# Autodesk Inventor assembly: 53
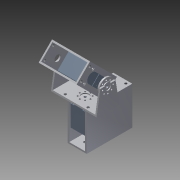
[picture p0: Inventor's stored thumbnail of the model, 180x180]
Saved by Autodesk Inventor 2013 (Build 170138000, 138)
## iProperties
Created: 2014-04-04
Part Number: 53
Document SubType Name: Assembly
Designer: andou
Author: andou
Title: Head
## Documents named in this file (7)
- C:\Users\andou\Documents\GitHub\Robotics-Project\design\RoboticsProject\project_4\Head.iam
- C:\Users\andou\Documents\GitHub\Robotics-Project\design\RoboticsProject\project_4\Long_Serial_Case.ipt
- C:\Users\andou\Documents\GitHub\Robotics-Project\design\RoboticsProject\project_4\Generic Parts\KRS-2542HV.ipt
- C:\Users\andou\Documents\GitHub\Robotics-Project\design\RoboticsProject\project_4\Generic Parts\Low_Height_Horn.ipt
- C:\Users\andou\Documents\GitHub\Robotics-Project\design\RoboticsProject\project_4\Complete_data\Bracket.ipt
- C:\Users\andou\Documents\GitHub\Robotics-Project\design\RoboticsProject\project_4\Complete_data\Serial_Case.ipt
- C:\Users\andou\Documents\GitHub\Robotics-Project\design\RoboticsProject\project_4\Complete_data\Free_Horn.iam
## Components (8 placed, 6 different names)
1. Long_Serial_Case:1 — 挿入:1, 挿入:2
2. KRS-2542HV:1 — 挿入:1, 挿入:2, 挿入:3
3. Low_Height_Horn:1 — 挿入:3, 挿入:7, 挿入:8
4. Bracket:1 — 挿入:7, 挿入:8, 挿入:10, 挿入:11, 挿入:12
5. Serial_Case:1 — 挿入:5, 挿入:6, 挿入:9
6. KRS-2542HV:2 — 挿入:4, 挿入:5, 挿入:6
7. Low_Height_Horn:2 — 挿入:4, 挿入:10, 挿入:11
8. Free_Horn:1 [sub-assembly] — 挿入:9, 挿入:12
## Relationships (12: Insert 12)
- 挿入:1 [Insert]: Long_Serial_Case:1 ↔ KRS-2542HV:1
- 挿入:2 [Insert]: Long_Serial_Case:1 ↔ KRS-2542HV:1
- 挿入:3 [Insert]: KRS-2542HV:1 ↔ Low_Height_Horn:1
- 挿入:4 [Insert]: KRS-2542HV:2 ↔ Low_Height_Horn:2
- 挿入:5 [Insert]: Serial_Case:1 ↔ KRS-2542HV:2
- 挿入:6 [Insert]: Serial_Case:1 ↔ KRS-2542HV:2
- 挿入:7 [Insert]: Low_Height_Horn:1 ↔ Bracket:1
- 挿入:8 [Insert]: Low_Height_Horn:1 ↔ Bracket:1
- 挿入:9 [Insert]: Serial_Case:1 ↔ Free_Horn:1
- 挿入:10 [Insert]: Bracket:1 ↔ Low_Height_Horn:2
- 挿入:11 [Insert]: Bracket:1 ↔ Low_Height_Horn:2
- 挿入:12 [Insert]: Bracket:1 ↔ Free_Horn:1
